# Autodesk Inventor assembly: dog_2
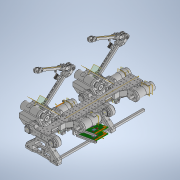
[picture p0: Inventor's stored thumbnail of the model, 180x180]
Saved by Autodesk Inventor 2020 (Build 240168000, 168)
## iProperties
Created: 2019-05-16
Part Number: dog_2
Document SubType Name: Assembly
Designer: psrob
Author: psrob
## Documents named in this file (3)
- E:\projects-2\project dog gen2\hardware\dog_2.iam
- E:\projects-2\project dog gen2\hardware\body_struct.iam
- E:\projects-2\project dog gen2\hardware\leg_bone_ass1.iam
## Components (3 placed, 2 different names)
1. body_struct:1 [sub-assembly] — Insert:1, Insert:2
2. leg_bone_ass1:1 [sub-assembly] — Insert:1
3. leg_bone_ass1:2 [sub-assembly] — Insert:2
## Relationships (2: Insert 2)
- Insert:1: body_struct:1 ↔ leg_bone_ass1:1
- Insert:2: body_struct:1 ↔ leg_bone_ass1:2
